# Autodesk Inventor assembly: recuperation
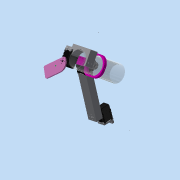
[picture p0: Inventor's stored thumbnail of the model, 180x180]
Saved by Autodesk Inventor 2017 (Build 210142000, 142)
## iProperties
Created: 2018-03-31
Part Number: recuperation
Document SubType Name: Assembly
Designer: franc
Mass: 446.753 g
Surface Area: 1710.63 cm^2
Volume: 446.753 cm^3
Density: 1 g/cm^3
Author: franc
## Documents named in this file (12)
- C:\Users\Aegir\Documents\robotik 2017\git\2018\robot\traitement-eau\recuperation.iam
- C:\Users\Aegir\Documents\robotik 2017\git\2018\robot\traitement-eau\cylindre-stockage.ipt
- C:\Users\Aegir\Documents\robotik 2017\git\composants\AX12\AX12.iam
- C:\Users\Aegir\Documents\robotik 2017\git\2018\robot\traitement-eau\trappe.ipt
- C:\Users\Aegir\Documents\robotik 2017\git\composants\AX12\F3.ipt
- C:\Users\Aegir\Documents\robotik 2017\git\2018\robot\traitement-eau\support-trappe.ipt
- C:\Users\Aegir\Documents\robotik 2017\git\composants\AX12\F2.ipt
- C:\Users\Aegir\Documents\robotik 2017\git\composants\AX12\ax12_wheel.ipt
- C:\Users\Aegir\Documents\robotik 2017\git\composants\AX12\ax12_box.ipt
- C:\Users\Aegir\Documents\robotik 2017\git\2018\robot\traitement-eau\rotation-recuperation.ipt
- C:\Users\Aegir\Documents\robotik 2017\git\2018\robot\traitement-eau\bras.ipt
- C:\Users\Aegir\Documents\robotik 2017\git\2018\robot\traitement-eau\fixation-bras.ipt
## Components (12 placed, 11 different names)
1. cylindre-stockage:1 — Affleurement:1, Tangente:7, Tangente:8, Tangente:9, Affleurement:3, Placage:22
2. AX12:1 [sub-assembly] — Affleurement:1, Tangente:5, Tangente:6, Placage:5, Placage:6, Placage:7, Placage:8, Tangente:7, Tangente:8
3. trappe:1 — Tangente:5, Tangente:6, Placage:5
4. F3:1 — Placage:6, Placage:7, Placage:8, Placage:9, Affleurement:2, Placage:10
5. support-trappe:1 — Placage:9, Affleurement:2, Placage:10, Affleurement:4
6. F2:1 — Placage:11, Placage:12, Placage:13, Tangente:9, Affleurement:3, Affleurement:4, Placage:14, Affleurement:5
7. ax12_wheel:1 — Placage:11, Placage:12, Placage:13
8. ax12_box:1 — Placage:15, Placage:16, Placage:17
9. rotation-recuperation:1 — Placage:14, Affleurement:5, Placage:22
10. bras:1 — Placage:15, Placage:16, Placage:17, Placage:18, Affleurement:6, Tangente:10
11. AX12:2 [sub-assembly] — Placage:18, Affleurement:6, Tangente:10, Placage:19, Placage:20, Placage:21
12. fixation-bras:1 — Placage:19, Placage:20, Placage:21
## Relationships (31: Mate 18, Flush 6, Tangent 6, Insert 1)
- Affleurement:1 [Flush]: cylindre-stockage:1 ↔ AX12:1
- Tangente:5: AX12:1 ↔ trappe:1
- Tangente:6: AX12:1 ↔ trappe:1
- Placage:5 [Mate]: AX12:1 ↔ trappe:1
- Placage:6 [Mate]: AX12:1 ↔ F3:1
- Placage:7 [Mate]: AX12:1 ↔ F3:1
- Placage:8 [Mate]: AX12:1 ↔ F3:1
- Tangente:7 (1 mm): cylindre-stockage:1 ↔ AX12:1
- Tangente:8: cylindre-stockage:1 ↔ AX12:1
- Placage:9 [Mate]: F3:1 ↔ support-trappe:1
- Affleurement:2 [Flush]: F3:1 ↔ support-trappe:1
- Placage:10 [Mate]: F3:1 ↔ support-trappe:1
- [Insert]: ax12_wheel:1 ↔ ax12_box:1
- Placage:11 [Mate]: F2:1 ↔ ax12_wheel:1
- Placage:12 [Mate]: F2:1 ↔ ax12_wheel:1
- Placage:13 [Mate]: F2:1 ↔ ax12_wheel:1
- Tangente:9 (1 mm): cylindre-stockage:1 ↔ F2:1
- Affleurement:3 [Flush] (87.5 mm): cylindre-stockage:1 ↔ F2:1
- Affleurement:4 [Flush] (25.5 mm): support-trappe:1 ↔ F2:1
- Placage:14 [Mate]: F2:1 ↔ rotation-recuperation:1
- Affleurement:5 [Flush]: F2:1 ↔ rotation-recuperation:1
- Placage:15 [Mate]: ax12_box:1 ↔ bras:1
- Placage:16 [Mate]: ax12_box:1 ↔ bras:1
- Placage:17 [Mate]: ax12_box:1 ↔ bras:1
- Placage:18 [Mate]: bras:1 ↔ AX12:2
- Affleurement:6 [Flush] (-23.5 mm): bras:1 ↔ AX12:2
- Tangente:10 (6 mm): bras:1 ↔ AX12:2
- Placage:19 [Mate]: AX12:2 ↔ fixation-bras:1
- Placage:20 [Mate]: AX12:2 ↔ fixation-bras:1
- Placage:21 [Mate]: AX12:2 ↔ fixation-bras:1
- Placage:22 [Mate]: cylindre-stockage:1 ↔ rotation-recuperation:1
## Named parameters: d28_d1 = 0 mm
